# Autodesk Inventor assembly: table_inter
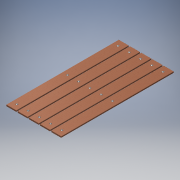
[picture p0: Inventor's stored thumbnail of the model, 180x180]
Saved by Autodesk Inventor 2019 (Build 230136000, 136)
## iProperties
Created: 2019-02-27
Part Number: table_inter
Document SubType Name: Assembly
Designer: gaincarlo
Author: gaincarlo
## Documents named in this file (4)
- D:\Giancarlo Bacchio\Documenti\00 - Progetti\30-Inventor\LaPanca-Baraca\table_inter.iam
- D:\Giancarlo Bacchio\Documenti\00 - Progetti\30-Inventor\LaPanca-Baraca\support1.ipt
- D:\Giancarlo Bacchio\Documenti\00 - Progetti\30-Inventor\LaPanca-Baraca\doga_interm.ipt
- D:\Giancarlo Bacchio\Documenti\Inventor\Content Center Files\R2019\en-US\GB_T 15-88\Bolt GB_T 15 M8 x 35.ipt
## Components (23 placed, 3 different names)
1. support1:2 — Mate:1, Mate:2, Angle:1
2. support1:3
3. support1:4
4. doga_interm:1 — Mate:1, Mate:2, Angle:1, Mate:3, Mate:4
5. doga_interm:2
6. doga_interm:3
7. doga_interm:4
8. doga_interm:5
9. Bolt GB/T 15-1988 M8x35:1 — Mate:3, Mate:4
10. Bolt GB/T 15-1988 M8x35:2
11. Bolt GB/T 15-1988 M8x35:3
12. Bolt GB/T 15-1988 M8x35:4
13. Bolt GB/T 15-1988 M8x35:5
14. Bolt GB/T 15-1988 M8x35:6
15. Bolt GB/T 15-1988 M8x35:7
16. Bolt GB/T 15-1988 M8x35:8
17. Bolt GB/T 15-1988 M8x35:9
18. Bolt GB/T 15-1988 M8x35:10
19. Bolt GB/T 15-1988 M8x35:11
20. Bolt GB/T 15-1988 M8x35:12
21. Bolt GB/T 15-1988 M8x35:13
22. Bolt GB/T 15-1988 M8x35:14
23. Bolt GB/T 15-1988 M8x35:15
## Component patterns: (3 elements, first: support1:2), (5 elements, first: doga_interm:1), (15 elements, first: Bolt GB/T 15-1988 M8x35:1)
## Relationships (5: Mate 4, Angle 1)
- Mate:1: support1:2 ↔ doga_interm:1
- Mate:2: support1:2 ↔ doga_interm:1
- Angle:1 (90 deg): support1:2 ↔ doga_interm:1
- Mate:3: doga_interm:1 ↔ Bolt GB/T 15-1988 M8x35:1
- Mate:4: doga_interm:1 ↔ Bolt GB/T 15-1988 M8x35:1
